# Autodesk Inventor assembly: WheelAssembly
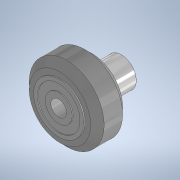
[picture p0: Inventor's stored thumbnail of the model, 180x180]
Saved by Autodesk Inventor 2022 (Build 260153000, 153)
## iProperties
Created: 2021-11-02
Part Number: WheelAssembly
Document SubType Name: Assembly
Designer: JK
Author: JK
## Documents named in this file (3)
- C:\Users\JK\Documents\Inventor\UTM\WheelAssembly.iam
- C:\Users\JK\Documents\Inventor\UTM\GantryPlateWheel.ipt
- C:\Users\JK\Documents\Inventor\UTM\9mmSpacer.ipt
## Components (2 placed, 2 different names)
1. GantryPlateWheel:1 — Coincidencia:1, Coincidencia:2
2. 9mmSpacer:1 — Coincidencia:1, Coincidencia:2
## Relationships (2: Mate 2)
- Coincidencia:1 [Mate]: GantryPlateWheel:1 ↔ 9mmSpacer:1
- Coincidencia:2 [Mate]: GantryPlateWheel:1 ↔ 9mmSpacer:1
